# Autodesk Inventor assembly: 하단 아크릴 조립품
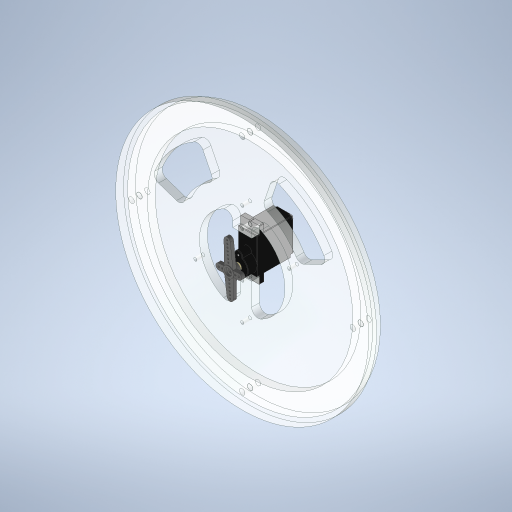
[picture p0: Inventor's stored thumbnail of the model, 512x512]
Saved by Autodesk Inventor 2023.1 (Build 271208000, 208)
## iProperties
Created: 2022-08-14
Part Number: 하단 아크릴 조립품
Document SubType Name: Assembly
Designer: fly01
Author: fly01
## Documents named in this file (5)
- C:\Users\fly01\Desktop\PAI설계 2\조림품\하단 아크릴 조립품.iam
- C:\Users\fly01\Desktop\PAI설계 2\출력품\아크릴 LED확산판.ipt
- C:\Users\fly01\Desktop\PAI설계 2\출력품\아크릴 고정판.ipt
- C:\Users\fly01\Desktop\PAI설계 2\범용 부품\180도 서보모터.ipt
- C:\Users\fly01\Desktop\PAI설계 2\범용 부품\180도 서보모터 십자축.ipt
## Components (4 placed, 4 different names)
1. 아크릴 LED확산판:1 — 삽입:1, 삽입:2, 삽입:3, 삽입:4
2. 아크릴 고정판:1 — 삽입:1, 삽입:2
3. 180도 서보모터:1 — 삽입:3, 삽입:4, 삽입:5
4. 180도 서보모터 십자축:1 — 삽입:5
## Relationships (5: Insert 5)
- 삽입:1 [Insert]: 아크릴 LED확산판:1 ↔ 아크릴 고정판:1
- 삽입:2 [Insert]: 아크릴 LED확산판:1 ↔ 아크릴 고정판:1
- 삽입:3 [Insert]: 아크릴 LED확산판:1 ↔ 180도 서보모터:1
- 삽입:4 [Insert]: 아크릴 LED확산판:1 ↔ 180도 서보모터:1
- 삽입:5 [Insert]: 180도 서보모터:1 ↔ 180도 서보모터 십자축:1
